# Autodesk Inventor assembly: bottomface
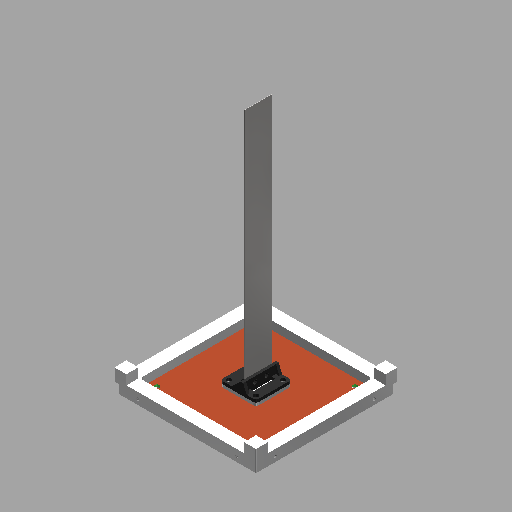
[picture p0: Inventor's stored thumbnail of the model, 512x512]
Saved by Autodesk Inventor 2022 (Build 260153000, 153)
## iProperties
Created: 2021-10-08
Part Number: bottomface
Document SubType Name: Assembly
Designer: Bowen O'Steen
Author: Bowen O'Steen
## Documents named in this file (6)
- C:\Users\gwhen\OneDrive\Desktop\Vault\Designs\MEMESat\MemeSat\Engineering Data\MemeSat\Assembly\FR-02assembled.iam
- C:\Users\gwhen\OneDrive\Desktop\Vault\Designs\MEMESat\MemeSat\Engineering Data\MemeSat\Frame\FR-02.ipt
- C:\Users\gwhen\OneDrive\Desktop\Vault\Designs\MEMESat\MemeSat\Engineering Data\MemeSat\Antenna\pcb.ipt
- C:\Users\gwhen\OneDrive\Desktop\Vault\Designs\MEMESat\MemeSat\Engineering Data\MemeSat\Antenna\connector.ipt
- C:\Users\gwhen\OneDrive\Desktop\Vault\Designs\MEMESat\MemeSat\Engineering Data\MemeSat\Antenna\antennabrace.ipt
- C:\Users\gwhen\OneDrive\Desktop\Vault\Designs\MEMESat\MemeSat\Engineering Data\MemeSat\Antenna\tape.ipt
## Components (5 placed, 5 different names)
1. FR-02:1 — Mate:1, Mate:2, Flush:1, Mate:4, Mate:5, Mate:16
2. pcb:1 — Mate:4, Mate:5, Mate:7, Mate:8, Mate:16, Mate:17
3. connector:1 — Mate:7, Mate:8, Mate:17, Mate:18, Mate:19, Mate:20
4. tape:1 — Mate:21, Mate:23, Mate:24
5. antennabrace:1 — Mate:18, Mate:19, Mate:20, Mate:21, Mate:23, Mate:24
## Relationships (15: Mate 14, Flush 1)
- Mate:1: FR-02:1
- Mate:2: FR-02:1
- Flush:1: FR-02:1
- Mate:4: FR-02:1 ↔ pcb:1
- Mate:5: FR-02:1 ↔ pcb:1
- Mate:7: pcb:1 ↔ connector:1
- Mate:8: pcb:1 ↔ connector:1
- Mate:16: FR-02:1 ↔ pcb:1
- Mate:17: pcb:1 ↔ connector:1
- Mate:18: connector:1 ↔ antennabrace:1
- Mate:19: connector:1 ↔ antennabrace:1
- Mate:20: connector:1 ↔ antennabrace:1
- Mate:21: tape:1 ↔ antennabrace:1
- Mate:23: tape:1 ↔ antennabrace:1
- Mate:24: tape:1 ↔ antennabrace:1
